# Autodesk Inventor assembly: Sheep
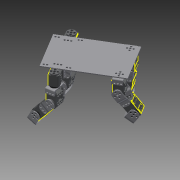
[picture p0: Inventor's stored thumbnail of the model, 180x180]
Saved by Autodesk Inventor 2014 SP1 (Build 180222100, 222)
## iProperties
Created: 2014-04-23
Part Number: Sheep
Document SubType Name: Assembly
Designer: david
Author: david
## Documents named in this file (7)
- C:\Users\asus\Documents\GitHub\SheepWarrior\Autodesk\V2\Sheep\Sheep.iam
- C:\Users\asus\Documents\GitHub\SheepWarrior\Autodesk\V2\Sheep\Body.ipt
- C:\Users\asus\Documents\GitHub\SheepWarrior\Autodesk\V2\Sheep\Equerre.ipt
- C:\Users\asus\Documents\GitHub\SheepWarrior\Autodesk\V2\XL320\src\Motor.iam
- C:\Users\asus\Documents\GitHub\SheepWarrior\Autodesk\V2\XL320\src\Pantilt.ipt
- C:\Users\asus\Documents\GitHub\SheepWarrior\Autodesk\V2\XL320\src\ArmToBottom.ipt
- C:\Users\asus\Documents\GitHub\SheepWarrior\Autodesk\V2\XL320\src\U.ipt
## Components (31 placed, 6 different names)
1. Body:1 — Mate:8, Mate:9, Mate:11, Mate:12, Mate:14, Mate:15, Mate:16, Mate:30, Mate:31, Mate:32, Mate:33, Mate:34, Mate:35, Mate:54, Mate:55, Mate:56, Mate:57, Mate:58, Mate:59, Mate:60, Mate:61, Mate:62
2. Equerre:1 — Mate:8, Mate:9
3. Equerre:2 — Mate:11, Mate:12
4. Motor:1 [sub-assembly] — Mate:14, Mate:15, Mate:16, Mate:17, Rotational:1
5. Pantilt:1 — Mate:17, Rotational:1, Mate:18, Mate:19, Mate:20
6. Motor:2 [sub-assembly] — Mate:18, Mate:19, Mate:20, Mate:21, Mate:24, Rotational:2, Rotational:3
7. ArmToBottom:1 — Mate:21, Rotational:3, Mate:25, Mate:26, Mate:27
8. ArmToBottom:2 — Mate:24, Rotational:2, Mate:28
9. Motor:3 [sub-assembly] — Mate:25, Mate:26, Mate:27, Mate:28, Mate:29, Rotational:4
10. U:1 — Mate:29, Rotational:4
11. Pantilt:2 — Mate:30, Mate:32, Mate:33, Mate:39, Mate:40, Mate:41
12. Pantilt:3 — Mate:31, Mate:34, Mate:35, Mate:36, Mate:37, Mate:38
13. Motor:4 [sub-assembly] — Mate:36, Mate:37, Mate:38, Mate:42, Rotational:5, Mate:43, Rotational:6
14. Motor:5 [sub-assembly] — Mate:44, Mate:45, Mate:46, Mate:53, Rotational:10
15. Motor:6 [sub-assembly] — Mate:39, Mate:40, Mate:41, Mate:47, Rotational:7, Mate:48, Rotational:8
16. Motor:7 [sub-assembly] — Mate:49, Mate:50, Mate:51, Mate:52, Rotational:9
17. ArmToBottom:3 — Mate:42, Rotational:5, Mate:44, Mate:45
18. ArmToBottom:4 — Mate:47, Rotational:7, Mate:51
19. ArmToBottom:5 — Mate:48, Rotational:8, Mate:49, Mate:50
20. ArmToBottom:6 — Mate:43, Rotational:6, Mate:46
21. U:2 — Mate:53, Rotational:10
22. U:3 — Mate:52, Rotational:9
23. Equerre:3 — Mate:54, Mate:58, Mate:59
24. Equerre:4 — Mate:55, Mate:56, Mate:57
25. Motor:8 [sub-assembly] — Mate:60, Mate:61, Mate:62, Mate:63, Rotational:11
26. Motor:9 [sub-assembly] — Mate:69, Mate:70, Mate:71, Mate:72, Rotational:14
27. Motor:10 [sub-assembly] — Mate:64, Mate:65, Mate:66, Mate:67, Rotational:12, Mate:68, Rotational:13
28. Pantilt:4 — Mate:63, Rotational:11, Mate:64, Mate:65, Mate:66
29. ArmToBottom:7 — Mate:67, Rotational:12, Mate:69, Mate:70
30. ArmToBottom:8 — Mate:68, Rotational:13, Mate:71
31. U:4 — Mate:72, Rotational:14
## Relationships (75: Mate 61, RevoluteJoint 14)
- Mate:8: Body:1 ↔ Equerre:1
- Mate:9: Body:1 ↔ Equerre:1
- Mate:11: Body:1 ↔ Equerre:2
- Mate:12: Body:1 ↔ Equerre:2
- Mate:14: Body:1 ↔ Motor:1
- Mate:15: Body:1 ↔ Motor:1
- Mate:16: Body:1 ↔ Motor:1
- Mate:17: Motor:1 ↔ Pantilt:1
- Rotational:1 [RevoluteJoint]: Motor:1 ↔ Pantilt:1
- Mate:18: Pantilt:1 ↔ Motor:2
- Mate:19: Pantilt:1 ↔ Motor:2
- Mate:20: Pantilt:1 ↔ Motor:2
- Mate:21: Motor:2 ↔ ArmToBottom:1
- Mate:24: Motor:2 ↔ ArmToBottom:2
- Rotational:2 [RevoluteJoint]: Motor:2 ↔ ArmToBottom:2
- Rotational:3 [RevoluteJoint]: Motor:2 ↔ ArmToBottom:1
- Mate:25: ArmToBottom:1 ↔ Motor:3
- Mate:26: ArmToBottom:1 ↔ Motor:3
- Mate:27: ArmToBottom:1 ↔ Motor:3
- Mate:28: ArmToBottom:2 ↔ Motor:3
- Mate:29: Motor:3 ↔ U:1
- Rotational:4 [RevoluteJoint]: Motor:3 ↔ U:1
- Mate:30: Body:1 ↔ Pantilt:2
- Mate:31: Body:1 ↔ Pantilt:3
- Mate:32: Body:1 ↔ Pantilt:2
- Mate:33: Body:1 ↔ Pantilt:2
- Mate:34: Body:1 ↔ Pantilt:3
- Mate:35: Body:1 ↔ Pantilt:3
- Mate:36: Pantilt:3 ↔ Motor:4
- Mate:37: Pantilt:3 ↔ Motor:4
- Mate:38: Pantilt:3 ↔ Motor:4
- Mate:39: Pantilt:2 ↔ Motor:6
- Mate:40: Pantilt:2 ↔ Motor:6
- Mate:41: Pantilt:2 ↔ Motor:6
- Mate:42: Motor:4 ↔ ArmToBottom:3
- Rotational:5 [RevoluteJoint]: Motor:4 ↔ ArmToBottom:3
- Mate:43: Motor:4 ↔ ArmToBottom:6
- Rotational:6 [RevoluteJoint]: Motor:4 ↔ ArmToBottom:6
- Mate:44: Motor:5 ↔ ArmToBottom:3
- Mate:45: Motor:5 ↔ ArmToBottom:3
- Mate:46: Motor:5 ↔ ArmToBottom:6
- Mate:47: Motor:6 ↔ ArmToBottom:4
- Rotational:7 [RevoluteJoint]: Motor:6 ↔ ArmToBottom:4
- Mate:48: Motor:6 ↔ ArmToBottom:5
- Rotational:8 [RevoluteJoint]: Motor:6 ↔ ArmToBottom:5
- Mate:49: Motor:7 ↔ ArmToBottom:5
- Mate:50: Motor:7 ↔ ArmToBottom:5
- Mate:51: Motor:7 ↔ ArmToBottom:4
- Mate:52: Motor:7 ↔ U:3
- Rotational:9 [RevoluteJoint]: Motor:7 ↔ U:3
- Mate:53: Motor:5 ↔ U:2
- Rotational:10 [RevoluteJoint]: Motor:5 ↔ U:2
- Mate:54: Body:1 ↔ Equerre:3
- Mate:55: Body:1 ↔ Equerre:4
- Mate:56: Body:1 ↔ Equerre:4
- Mate:57: Body:1 ↔ Equerre:4
- Mate:58: Body:1 ↔ Equerre:3
- Mate:59: Body:1 ↔ Equerre:3
- Mate:60: Body:1 ↔ Motor:8
- Mate:61: Body:1 ↔ Motor:8
- Mate:62: Body:1 ↔ Motor:8
- Mate:63: Motor:8 ↔ Pantilt:4
- Rotational:11 [RevoluteJoint]: Motor:8 ↔ Pantilt:4
- Mate:64: Motor:10 ↔ Pantilt:4
- Mate:65: Motor:10 ↔ Pantilt:4
- Mate:66: Motor:10 ↔ Pantilt:4
- Mate:67: Motor:10 ↔ ArmToBottom:7
- Rotational:12 [RevoluteJoint]: Motor:10 ↔ ArmToBottom:7
- Mate:68: Motor:10 ↔ ArmToBottom:8
- Rotational:13 [RevoluteJoint]: Motor:10 ↔ ArmToBottom:8
- Mate:69: Motor:9 ↔ ArmToBottom:7
- Mate:70: Motor:9 ↔ ArmToBottom:7
- Mate:71: Motor:9 ↔ ArmToBottom:8
- Mate:72: Motor:9 ↔ U:4
- Rotational:14 [RevoluteJoint]: Motor:9 ↔ U:4
